# Autodesk Inventor assembly: S8x2
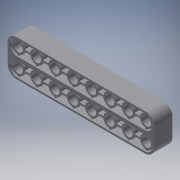
[picture p0: Inventor's stored thumbnail of the model, 180x180]
Saved by Autodesk Inventor 2019 (Build 230136000, 136)
## iProperties
Created: 2019-01-31
Part Number: S8x2
Document SubType Name: Assembly
Designer: Varga Daniel
Author: Varga Daniel
## Documents named in this file (3)
- C:\!_Dani\!_cloud\OneDrive\!_munka\Revolution\RevvyDemoKit\Structural parts\Straight Beams\S8x2.iam
- C:\!_Dani\!_cloud\OneDrive\!_munka\Revolution\RevvyDemoKit\Structural parts\Straight Beams\straight_beam_end_part_double.ipt
- C:\!_Dani\!_cloud\OneDrive\!_munka\Revolution\RevvyDemoKit\Structural parts\Straight Beams\straight_beam_inner_part_double.ipt
## Components (8 placed, 2 different names)
1. straight_beam_end_part_double:1 — Flush:8, Flush:9, Mate:2
2. straight_beam_end_part_double:2 — Flush:6, Mate:1, Flush:7
3. straight_beam_inner_part_double:1 — Flush:3, Flush:4, Flush:12, Flush:13, Mate:5, Mate:6
4. straight_beam_inner_part_double:2 — Flush:4, Flush:5, Flush:13, Flush:14, Mate:6, Mate:7
5. straight_beam_inner_part_double:3 — Flush:5, Flush:6, Mate:1, Flush:7, Flush:14, Mate:7
6. straight_beam_inner_part_double:4 — Flush:2, Flush:3, Flush:11, Flush:12, Mate:4, Mate:5
7. straight_beam_inner_part_double:5 — Flush:1, Flush:2, Flush:10, Flush:11, Mate:3, Mate:4
8. straight_beam_inner_part_double:6 — Flush:1, Flush:8, Flush:9, Mate:2, Flush:10, Mate:3
## Relationships (21: Flush 14, Mate 7)
- Flush:1: straight_beam_inner_part_double:5 ↔ straight_beam_inner_part_double:6
- Flush:2: straight_beam_inner_part_double:4 ↔ straight_beam_inner_part_double:5
- Flush:3: straight_beam_inner_part_double:1 ↔ straight_beam_inner_part_double:4
- Flush:4: straight_beam_inner_part_double:1 ↔ straight_beam_inner_part_double:2
- Flush:5: straight_beam_inner_part_double:2 ↔ straight_beam_inner_part_double:3
- Flush:6: straight_beam_end_part_double:2 ↔ straight_beam_inner_part_double:3
- Mate:1: straight_beam_end_part_double:2 ↔ straight_beam_inner_part_double:3
- Flush:7: straight_beam_end_part_double:2 ↔ straight_beam_inner_part_double:3
- Flush:8: straight_beam_end_part_double:1 ↔ straight_beam_inner_part_double:6
- Flush:9: straight_beam_end_part_double:1 ↔ straight_beam_inner_part_double:6
- Mate:2: straight_beam_end_part_double:1 ↔ straight_beam_inner_part_double:6
- Flush:10: straight_beam_inner_part_double:5 ↔ straight_beam_inner_part_double:6
- Flush:11: straight_beam_inner_part_double:4 ↔ straight_beam_inner_part_double:5
- Flush:12: straight_beam_inner_part_double:1 ↔ straight_beam_inner_part_double:4
- Flush:13: straight_beam_inner_part_double:1 ↔ straight_beam_inner_part_double:2
- Flush:14: straight_beam_inner_part_double:2 ↔ straight_beam_inner_part_double:3
- Mate:3: straight_beam_inner_part_double:5 ↔ straight_beam_inner_part_double:6
- Mate:4: straight_beam_inner_part_double:4 ↔ straight_beam_inner_part_double:5
- Mate:5: straight_beam_inner_part_double:1 ↔ straight_beam_inner_part_double:4
- Mate:6: straight_beam_inner_part_double:1 ↔ straight_beam_inner_part_double:2
- Mate:7: straight_beam_inner_part_double:2 ↔ straight_beam_inner_part_double:3
